# Autodesk Inventor assembly: derive_rod_v7
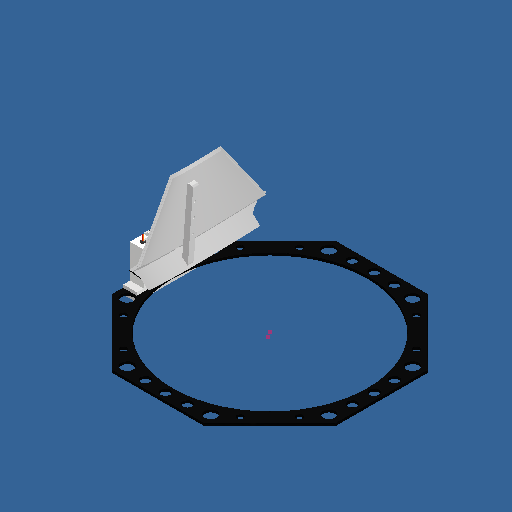
[picture p0: Inventor's stored thumbnail of the model, 512x512]
Saved by Autodesk Inventor 2026.2 (Build 302298000, 298)
## iProperties
Created: 2026-01-13
Part Number: derive_rod_v7
Document SubType Name: Assembly
Designer: Thoma
Author: Thoma
## Documents named in this file (10)
- C:\Users\Thoma\OneDrive\Desktop\dir\telescope_cover\cover\derive_base_plate_v5.2.iam
- C:\Users\Thoma\OneDrive\Desktop\dir\telescope_cover\telescope\version_3\Telescope_End.ipt
- C:\Users\Thoma\OneDrive\Desktop\dir\telescope_cover\cover\Cover_Upper_v3.ipt
- C:\Users\Thoma\OneDrive\Desktop\dir\telescope_cover\servo\DSS-M15S Servo.ipt
- C:\Users\Thoma\OneDrive\Desktop\dir\telescope_cover\cover\rod_v10.ipt
- C:\Users\Thoma\OneDrive\Desktop\dir\telescope_cover\cover\base_plate_v4.ipt
- C:\Users\Thoma\OneDrive\Desktop\dir\telescope_cover\cover\Base_Plate_bottom.ipt
- C:\Users\Thoma\OneDrive\Desktop\dir\telescope_cover\cover\4mm_screw.ipt
- C:\Users\Thoma\OneDrive\Desktop\dir\telescope_cover\cover\8mm_washer_1mm.ipt
- C:\Users\Thoma\OneDrive\Desktop\dir\telescope_cover\cover\derive_base_plate_v5.1.ipt
## Components (16 placed, 9 different names)
1. Telescope_End:1 — Flush:1, Mate:19, Mate:20, Mate:21, Mate:24
2. Cover_Upper_v3:1 — Mate:15, Mate:16, Tangent:1
3. DSS-M15S Servo:1 — Flush:1, Mate:17, Mate:18, Mate:22, Mate:23, Angle:3
4. rod_v10:1 — Mate:15, Mate:16, Tangent:1, Mate:17, Mate:18, Mate:44
5. base_plate_v4:1 — Mate:19, Mate:20, Mate:21, Mate:22, Mate:23, Flush:3, Flush:2, Angle:2, Mate:27, Mate:28, Mate:29, Mate:31, Mate:32, Mate:33, Mate:35, Mate:36, Mate:37, Mate:39, Mate:40, Mate:41, Flush:4, Mate:43
6. Base_Plate_bottom:1 — Mate:24, Flush:2, Flush:3, Mate:25, Mate:26, Angle:1
7. 4mm_screw:1 — Mate:25, Mate:26, Angle:1
8. 8mm_washer_1mm:1 — Angle:2, Mate:27, Mate:28, Mate:30
9. 4mm_screw:2 — Mate:29, Mate:30, Angle:3
10. 4mm_screw:3 — Mate:33, Mate:34
11. 4mm_screw:4 — Mate:41, Mate:42
12. 4mm_screw:5 — Mate:37, Mate:38
13. 8mm_washer_1mm:2 — Mate:35, Mate:36, Mate:38
14. 8mm_washer_1mm:3 — Mate:39, Mate:40, Mate:42
15. 8mm_washer_1mm:4 — Mate:31, Mate:32, Mate:34
16. derive_base_plate_v5.1:1 — Flush:4, Mate:43, Mate:44
## Relationships (38: Mate 30, Flush 4, Angle 3, Tangent 1)
- Flush:1 (2.5 mm): Telescope_End:1 ↔ DSS-M15S Servo:1
- Mate:15: Cover_Upper_v3:1 ↔ rod_v10:1
- Mate:16: Cover_Upper_v3:1 ↔ rod_v10:1
- Tangent:1 (-1 mm): Cover_Upper_v3:1 ↔ rod_v10:1
- Mate:17: DSS-M15S Servo:1 ↔ rod_v10:1
- Mate:18: DSS-M15S Servo:1 ↔ rod_v10:1
- Mate:19: Telescope_End:1 ↔ base_plate_v4:1
- Mate:20: Telescope_End:1 ↔ base_plate_v4:1
- Mate:21: Telescope_End:1 ↔ base_plate_v4:1
- Mate:22 (1.1 mm): DSS-M15S Servo:1 ↔ base_plate_v4:1
- Mate:23: DSS-M15S Servo:1 ↔ base_plate_v4:1
- Mate:24: Telescope_End:1 ↔ Base_Plate_bottom:1
- Flush:2: base_plate_v4:1 ↔ Base_Plate_bottom:1
- Flush:3: base_plate_v4:1 ↔ Base_Plate_bottom:1
- Mate:25: Base_Plate_bottom:1 ↔ 4mm_screw:1
- Mate:26: Base_Plate_bottom:1 ↔ 4mm_screw:1
- Angle:1 (0 deg): Base_Plate_bottom:1 ↔ 4mm_screw:1
- Angle:2 (0 deg): base_plate_v4:1 ↔ 8mm_washer_1mm:1
- Mate:27: base_plate_v4:1 ↔ 8mm_washer_1mm:1
- Mate:28: base_plate_v4:1 ↔ 8mm_washer_1mm:1
- Mate:29: base_plate_v4:1 ↔ 4mm_screw:2
- Mate:30: 8mm_washer_1mm:1 ↔ 4mm_screw:2
- Angle:3 (0 deg): DSS-M15S Servo:1 ↔ 4mm_screw:2
- Mate:31: base_plate_v4:1 ↔ 8mm_washer_1mm:4
- Mate:32: base_plate_v4:1 ↔ 8mm_washer_1mm:4
- Mate:33: base_plate_v4:1 ↔ 4mm_screw:3
- Mate:34: 4mm_screw:3 ↔ 8mm_washer_1mm:4
- Mate:35: base_plate_v4:1 ↔ 8mm_washer_1mm:2
- Mate:36: base_plate_v4:1 ↔ 8mm_washer_1mm:2
- Mate:37: base_plate_v4:1 ↔ 4mm_screw:5
- Mate:38: 4mm_screw:5 ↔ 8mm_washer_1mm:2
- Mate:39: base_plate_v4:1 ↔ 8mm_washer_1mm:3
- Mate:40: base_plate_v4:1 ↔ 8mm_washer_1mm:3
- Mate:41: base_plate_v4:1 ↔ 4mm_screw:4
- Mate:42: 4mm_screw:4 ↔ 8mm_washer_1mm:3
- Flush:4 (3.5 mm): base_plate_v4:1 ↔ derive_base_plate_v5.1:1
- Mate:43: base_plate_v4:1 ↔ derive_base_plate_v5.1:1
- Mate:44: rod_v10:1 ↔ derive_base_plate_v5.1:1
